# Autodesk Inventor assembly: ResistojetPrototype
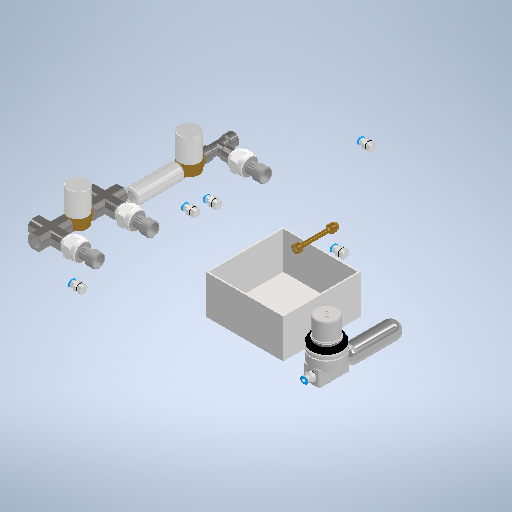
[picture p0: Inventor's stored thumbnail of the model, 512x512]
Saved by Autodesk Inventor 2025.2 (Build 292293000, 293)
## iProperties
Created: 2026-06-11
Part Number: ResistojetPrototype
Document SubType Name: Assembly
Designer: Simon
Author: Simon
## Documents named in this file (12)
- C:\Users\Simon\Projects\MEng Electronics\Development of a Resistojet Thruster\3) Hardware\Resistojet Design\Prototype Design\ResistojetPrototype.iam
- C:\Users\Simon\Projects\MEng Electronics\Development of a Resistojet Thruster\3) Hardware\Resistojet Design\Prototype Design\Heater.ipt
- C:\Users\Simon\Projects\MEng Electronics\Development of a Resistojet Thruster\3) Hardware\Resistojet Design\Prototype Design\0.4 nozzle.ipt
- C:\Users\Simon\Projects\MEng Electronics\Development of a Resistojet Thruster\3) Hardware\Resistojet Design\Prototype Design\PressureSensor.ipt
- C:\Users\Simon\Projects\MEng Electronics\Development of a Resistojet Thruster\3) Hardware\Resistojet Design\Prototype Design\SolenoidValve.ipt
- C:\Users\Simon\Projects\MEng Electronics\Development of a Resistojet Thruster\3) Hardware\Resistojet Design\Prototype Design\Plenum.ipt
- C:\Users\Simon\Projects\MEng Electronics\Development of a Resistojet Thruster\3) Hardware\Resistojet Design\Prototype Design\0,250' NPT TEE.ipt
- C:\Users\Simon\Projects\MEng Electronics\Development of a Resistojet Thruster\3) Hardware\Resistojet Design\Prototype Design\1-4 NPT 4 Way Cross Pneumatic Fitting.ipt
- C:\Users\Simon\Projects\MEng Electronics\Development of a Resistojet Thruster\3) Hardware\Resistojet Design\Prototype Design\AP100-02\AP100-F02.iam
- C:\Users\Simon\Projects\MEng Electronics\Development of a Resistojet Thruster\3) Hardware\Resistojet Design\Prototype Design\BicycleTank.ipt
- C:\Users\Simon\Projects\MEng Electronics\Development of a Resistojet Thruster\3) Hardware\Resistojet Design\Prototype Design\Festo_Pneumatic_Coupling_PC4-M10.ipt
- C:\Users\Simon\Projects\MEng Electronics\Development of a Resistojet Thruster\3) Hardware\Resistojet Design\Prototype Design\Box.ipt
## Components (20 placed, 11 different names)
1. Heater:1 — Mate:31, Mate:32
2. 0.4 nozzle:1 — Mate:31, Mate:32
3. PressureSensor:1 — Mate:16, Mate:25
4. PressureSensor:2 — Mate:6, Mate:8
5. PressureSensor:3 — Mate:19, Mate:26
6. SolenoidValve:1 — Mate:5, Flush:1, Mate:7, Mate:9, Mate:10
7. SolenoidValve:2 — Flush:1, Mate:15, Mate:18, Mate:23, Mate:24
8. Plenum:1 — Mate:9, Mate:10
9. 0,250' NPT TEE:1 — Mate:5, Mate:6, Mate:7, Mate:8
10. 1-4 NPT 4 Way Cross Pneumatic Fitting:1 — Mate:15, Mate:16, Mate:24, Mate:25
11. 1-4 NPT 4 Way Cross Pneumatic Fitting:2 — Mate:18, Mate:19, Mate:23, Mate:26
12. AP100-F02:1 [sub-assembly] — Mate:27, Mate:28, Mate:29, Mate:30
13. BicycleTank:1 — Mate:27, Mate:29
14. Festo_Pneumatic_Coupling_PC4-M10:1
15. Festo_Pneumatic_Coupling_PC4-M10:2
16. Festo_Pneumatic_Coupling_PC4-M10:3
17. Festo_Pneumatic_Coupling_PC4-M10:4
18. Festo_Pneumatic_Coupling_PC4-M10:5
19. Festo_Pneumatic_Coupling_PC4-M10:6 — Mate:28, Mate:30
20. Box:1
## Relationships (21: Mate 20, Flush 1)
- Mate:5: SolenoidValve:1 ↔ 0,250' NPT TEE:1
- Mate:6: PressureSensor:2 ↔ 0,250' NPT TEE:1
- Flush:1: SolenoidValve:1 ↔ SolenoidValve:2
- Mate:7 (-10 mm): SolenoidValve:1 ↔ 0,250' NPT TEE:1
- Mate:8 (-7 mm): PressureSensor:2 ↔ 0,250' NPT TEE:1
- Mate:9: SolenoidValve:1 ↔ Plenum:1
- Mate:10 (-10 mm): SolenoidValve:1 ↔ Plenum:1
- Mate:15: SolenoidValve:2 ↔ 1-4 NPT 4 Way Cross Pneumatic Fitting:1
- Mate:16: PressureSensor:1 ↔ 1-4 NPT 4 Way Cross Pneumatic Fitting:1
- Mate:18: SolenoidValve:2 ↔ 1-4 NPT 4 Way Cross Pneumatic Fitting:2
- Mate:19: PressureSensor:3 ↔ 1-4 NPT 4 Way Cross Pneumatic Fitting:2
- Mate:23 (-10 mm): SolenoidValve:2 ↔ 1-4 NPT 4 Way Cross Pneumatic Fitting:2
- Mate:24 (-10 mm): SolenoidValve:2 ↔ 1-4 NPT 4 Way Cross Pneumatic Fitting:1
- Mate:25 (-7 mm): PressureSensor:1 ↔ 1-4 NPT 4 Way Cross Pneumatic Fitting:1
- Mate:26 (-7 mm): PressureSensor:3 ↔ 1-4 NPT 4 Way Cross Pneumatic Fitting:2
- Mate:27: AP100-F02:1 ↔ BicycleTank:1
- Mate:28: AP100-F02:1 ↔ Festo_Pneumatic_Coupling_PC4-M10:6
- Mate:29 (-15 mm): AP100-F02:1 ↔ BicycleTank:1
- Mate:30 (-6 mm): AP100-F02:1 ↔ Festo_Pneumatic_Coupling_PC4-M10:6
- Mate:31: Heater:1 ↔ 0.4 nozzle:1
- Mate:32: Heater:1 ↔ 0.4 nozzle:1
